# Autodesk Inventor assembly: Assembly1
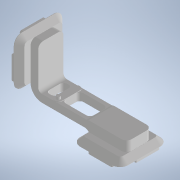
[picture p0: Inventor's stored thumbnail of the model, 180x180]
Saved by Autodesk Inventor 2020.2 (Build 242310000, 310)
## iProperties
Created: 2020-03-04
Part Number: Assembly1
Document SubType Name: Assembly
Designer: Kjell
Author: Kjell
## Documents named in this file (4)
- C:\Users\Kjell\Documents\Inventor\Fuji_X-T3_Lplate\Assembly1.iam
- C:\Users\Kjell\Documents\Inventor\Fuji_X-T3_Lplate\Dovetail.ipt
- C:\Users\Kjell\Documents\Inventor\Fuji_X-T3_Lplate\LBody.ipt
- C:\Users\Kjell\Documents\Inventor\Fuji_X-T3_Lplate\master_sketch.ipt
## Components (4 placed, 3 different names)
1. master_sketch:1
2. Dovetail:1 — Mate:1, Mate:2
3. LBody:1 — Mate:1, Mate:2, Mate:3, Mate:4
4. Dovetail:2 — Mate:3, Mate:4
## Relationships (4: Mate 4)
- Mate:1: Dovetail:1 ↔ LBody:1
- Mate:2: Dovetail:1 ↔ LBody:1
- Mate:3: LBody:1 ↔ Dovetail:2
- Mate:4: LBody:1 ↔ Dovetail:2
